# Autodesk Inventor assembly: Turret ASM
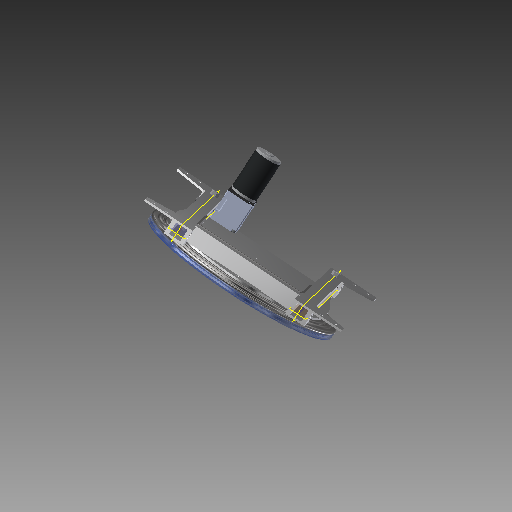
[picture p0: Inventor's stored thumbnail of the model, 512x512]
Saved by Autodesk Inventor 2017 (Build 210142000, 142)
## iProperties
Created: 2016-09-26
Part Number: Turret ASM
Document SubType Name: Assembly
Designer: Hanson
Author: Hanson
## Documents named in this file (19)
- C:\Users\Thariq\Documents\GitHub\bps-bunnybots2016-cad\bps-bunnybots2016-cad\Bunnybot-To_be_renamed\15102898-16-A-0000\15102898-16-A-0600\Turret ASM.iam
- C:\Users\Thariq\Documents\GitHub\bps-bunnybots2016-cad\bps-bunnybots2016-cad\Bunnybot-To_be_renamed\15102898-16-A-0000\15102898-16-A-0600\User Library-LazySusan 12inch.ipt
- C:\Users\Thariq\Documents\GitHub\bps-bunnybots2016-cad\bps-bunnybots2016-cad\Bunnybot-To_be_renamed\15102898-16-A-0000\15102898-16-A-0600\Large crossbeam.ipt
- C:\Users\Thariq\Documents\GitHub\bps-bunnybots2016-cad\bps-bunnybots2016-cad\Bunnybot-To_be_renamed\15102898-16-A-0000\15102898-16-A-0600\90480A195_LOW-STRENGTH STEEL HEX NUT.ipt
- C:\Users\Thariq\Documents\GitHub\bps-bunnybots2016-cad\bps-bunnybots2016-cad\Bunnybot-To_be_renamed\15102898-16-A-0000\15102898-16-A-0600\92196A277_18-8 STAINLESS STEEL SOCKET HEAD CAP SCREW.ipt
- C:\Users\Thariq\Documents\GitHub\bps-bunnybots2016-cad\bps-bunnybots2016-cad\Bunnybot-To_be_renamed\15102898-16-A-0000\15102898-16-A-0600\BAG motor top plate.ipt
- C:\Users\Thariq\Documents\GitHub\bps-bunnybots2016-cad\bps-bunnybots2016-cad\Bunnybot-To_be_renamed\15102898-16-A-0000\15102898-16-A-0600\92196A545_18-8 STAINLESS STEEL SOCKET HEAD CAP SCREW.ipt
- C:\Users\Thariq\Documents\GitHub\bps-bunnybots2016-cad\bps-bunnybots2016-cad\Bunnybot-To_be_renamed\15102898-16-A-0000\15102898-16-A-0600\plate mount nut.ipt
- C:\Users\Thariq\Documents\GitHub\bps-bunnybots2016-cad\bps-bunnybots2016-cad\Bunnybot-To_be_renamed\15102898-16-A-0000\15102898-16-A-0600\lazy susan bushing.ipt
- C:\Users\Thariq\Documents\GitHub\bps-bunnybots2016-cad\bps-bunnybots2016-cad\Bunnybot-To_be_renamed\15102898-16-A-0000\15102898-16-A-0600\BAG motor\VersaPlanetary-1-Stage-with-BAG-Motor.iam
- C:\Users\Thariq\Documents\GitHub\bps-bunnybots2016-cad\bps-bunnybots2016-cad\Bunnybot-To_be_renamed\15102898-16-A-0000\15102898-16-A-0600\217-2642-STEP-20140807.ipt
- C:\Users\Thariq\Documents\GitHub\bps-bunnybots2016-cad\bps-bunnybots2016-cad\Bunnybot-To_be_renamed\15102898-16-A-0000\15102898-16-A-0600\support ring.ipt
- C:\Users\Thariq\Documents\GitHub\bps-bunnybots2016-cad\bps-bunnybots2016-cad\Bunnybot-To_be_renamed\15102898-16-A-0000\15102898-16-A-0600\roundplate.ipt
- C:\Users\Thariq\Documents\GitHub\bps-bunnybots2016-cad\bps-bunnybots2016-cad\Bunnybot-To_be_renamed\15102898-16-A-0000\15102898-16-A-0600\Turret ASM\Design Accelerator\Chain Drive3.iam
- C:\Users\Thariq\Documents\GitHub\bps-bunnybots2016-cad\bps-bunnybots2016-cad\Bunnybot-To_be_renamed\15102898-16-A-0000\15102898-16-A-0200\Imported Components\1556A170_BRACKET.ipt
- C:\Users\Thariq\Documents\GitHub\bps-bunnybots2016-cad\bps-bunnybots2016-cad\Bunnybot-To_be_renamed\15102898-16-A-0000\15102898-16-A-0600\horizontal bar.ipt
- C:\Users\Thariq\Documents\GitHub\bps-bunnybots2016-cad\bps-bunnybots2016-cad\Bunnybot-To_be_renamed\15102898-16-A-0000\15102898-16-A-0600\2x1 angle bracket.ipt
- C:\Users\Thariq\Documents\GitHub\bps-bunnybots2016-cad\bps-bunnybots2016-cad\Bunnybot-To_be_renamed\15102898-16-A-0000\15102898-16-A-0600\15102898-16-P-0207.ipt
- C:\Users\Thariq\Documents\GitHub\bps-bunnybots2016-cad\bps-bunnybots2016-cad\Bunnybot-To_be_renamed\15102898-16-A-0000\15102898-16-A-0600\15102898-16-P-0208.ipt
## Components (27 placed, 18 different names)
1. User Library-LazySusan 12inch:1 — Mate:5, Mate:7, Mate:10, Mate:25, Mate:26, Mate:27, Mate:28, Mate:29
2. Large crossbeam:1 — Insert:16, Flush:1, Flush:2, Mate:17, Flush:3, Mate:34, Mate:35, Flush:10, Mate:41, Flush:14, Flush:17, Mate:43, Flush:18, Mate:44, Flush:19, Flush:20
3. Large crossbeam:2 — Insert:13, Insert:14, Insert:15, Flush:1, Mate:14, Flush:2, Mate:19, Flush:6, Flush:8, Flush:9, Mate:37, Flush:11, Mate:39, Flush:12, Mate:42, Flush:15, Flush:16, Flush:21, Mate:45, Flush:22
4. 92196A277_18-8 STAINLESS STEEL SOCKET HEAD CAP SCREW:1 — Insert:13
5. 92196A277_18-8 STAINLESS STEEL SOCKET HEAD CAP SCREW:2 — Insert:14
6. BAG motor top plate:1 — Insert:11, Insert:12, Mate:14, Flush:3, Mate:18, Flush:4, Flush:6, Mate:25, Mate:26, Mate:27, Mate:30
7. 92196A545_18-8 STAINLESS STEEL SOCKET HEAD CAP SCREW:1 — Insert:11
8. 92196A545_18-8 STAINLESS STEEL SOCKET HEAD CAP SCREW:2 — Insert:12, Mate:17
9. plate mount nut:1 — Insert:15
10. plate mount nut:2 — Insert:16
11. lazy susan bushing:1 — Mate:5, Mate:24
12. 90480A195_LOW-STRENGTH STEEL HEX NUT:2 — Mate:7, Mate:24
13. 90480A195_LOW-STRENGTH STEEL HEX NUT:4 — Mate:10
14. VersaPlanetary-1-Stage-with-BAG-Motor:1 [sub-assembly] — Mate:18, Mate:19, Flush:4, Mate:20, Mate:21
15. 217-2642-STEP-20140807:1 — Mate:20, Mate:21, Flush:7
16. support ring:1 — Mate:28, Mate:29, Mate:30, Mate:31, Mate:32, Mate:33
17. roundplate:1 — Mate:31, Mate:32, Mate:33, Flush:7
18. Chain Drive:1 [sub-assembly]
19. 1556A170_BRACKET:1 — Mate:37, Mate:38, Flush:11
20. 1556A170_BRACKET:2 — Mate:35, Mate:36, Flush:10
21. horizontal bar:1 — Mate:34, Flush:8, Flush:9, Mate:36, Mate:38, Mate:40
22. 2x1 angle bracket:1 — Mate:39, Mate:40, Flush:12, Flush:13
23. 2x1 angle bracket:2 — Flush:13, Mate:41, Flush:14
24. 15102898-16-P-0207:1 — Flush:17, Mate:43, Flush:18
25. 15102898-16-P-0208:1 — Mate:42, Flush:15, Flush:16
26. 15102898-16-P-0207:2 — Flush:21, Mate:45, Flush:22
27. 15102898-16-P-0208:2 — Mate:44, Flush:19, Flush:20
## Relationships (58: Mate 31, Flush 21, Insert 6)
- Insert:11: BAG motor top plate:1 ↔ 92196A545_18-8 STAINLESS STEEL SOCKET HEAD CAP SCREW:1
- Insert:12: BAG motor top plate:1 ↔ 92196A545_18-8 STAINLESS STEEL SOCKET HEAD CAP SCREW:2
- Insert:13: Large crossbeam:2 ↔ 92196A277_18-8 STAINLESS STEEL SOCKET HEAD CAP SCREW:1
- Insert:14: Large crossbeam:2 ↔ 92196A277_18-8 STAINLESS STEEL SOCKET HEAD CAP SCREW:2
- Insert:15: Large crossbeam:2 ↔ plate mount nut:1
- Insert:16: Large crossbeam:1 ↔ plate mount nut:2
- Flush:1: Large crossbeam:1 ↔ Large crossbeam:2
- Mate:5: User Library-LazySusan 12inch:1 ↔ lazy susan bushing:1
- Mate:7: User Library-LazySusan 12inch:1 ↔ 90480A195_LOW-STRENGTH STEEL HEX NUT:2
- Mate:10: User Library-LazySusan 12inch:1 ↔ 90480A195_LOW-STRENGTH STEEL HEX NUT:4
- Mate:14: Large crossbeam:2 ↔ BAG motor top plate:1
- Flush:2: Large crossbeam:1 ↔ Large crossbeam:2
- Mate:17: Large crossbeam:1 ↔ 92196A545_18-8 STAINLESS STEEL SOCKET HEAD CAP SCREW:2
- Flush:3: Large crossbeam:1 ↔ BAG motor top plate:1
- Mate:18: BAG motor top plate:1 ↔ VersaPlanetary-1-Stage-with-BAG-Motor:1
- Mate:19: Large crossbeam:2 ↔ VersaPlanetary-1-Stage-with-BAG-Motor:1
- Flush:4: BAG motor top plate:1 ↔ VersaPlanetary-1-Stage-with-BAG-Motor:1
- Mate:20: VersaPlanetary-1-Stage-with-BAG-Motor:1 ↔ 217-2642-STEP-20140807:1
- Mate:21: VersaPlanetary-1-Stage-with-BAG-Motor:1 ↔ 217-2642-STEP-20140807:1
- Mate:24: lazy susan bushing:1 ↔ 90480A195_LOW-STRENGTH STEEL HEX NUT:2
- Flush:6: Large crossbeam:2 ↔ BAG motor top plate:1
- Mate:25: User Library-LazySusan 12inch:1 ↔ BAG motor top plate:1
- Mate:26: User Library-LazySusan 12inch:1 ↔ BAG motor top plate:1
- Mate:27: User Library-LazySusan 12inch:1 ↔ BAG motor top plate:1
- Mate:28: User Library-LazySusan 12inch:1 ↔ support ring:1
- Mate:29: User Library-LazySusan 12inch:1 ↔ support ring:1
- Mate:30: BAG motor top plate:1 ↔ support ring:1
- Mate:31: support ring:1 ↔ roundplate:1
- Mate:32: support ring:1 ↔ roundplate:1
- Mate:33: support ring:1 ↔ roundplate:1
- Flush:7: 217-2642-STEP-20140807:1 ↔ roundplate:1
- Mate:34: Large crossbeam:1 ↔ horizontal bar:1
- Flush:8: Large crossbeam:2 ↔ horizontal bar:1
- Flush:9 (50.8 mm): Large crossbeam:2 ↔ horizontal bar:1
- Mate:35: Large crossbeam:1 ↔ 1556A170_BRACKET:2
- Mate:36: 1556A170_BRACKET:2 ↔ horizontal bar:1
- Flush:10: Large crossbeam:1 ↔ 1556A170_BRACKET:2
- Mate:37: Large crossbeam:2 ↔ 1556A170_BRACKET:1
- Mate:38: 1556A170_BRACKET:1 ↔ horizontal bar:1
- Flush:11: Large crossbeam:2 ↔ 1556A170_BRACKET:1
- Mate:39: Large crossbeam:2 ↔ 2x1 angle bracket:1
- Mate:40: horizontal bar:1 ↔ 2x1 angle bracket:1
- Flush:12: Large crossbeam:2 ↔ 2x1 angle bracket:1
- Flush:13: 2x1 angle bracket:1 ↔ 2x1 angle bracket:2
- Mate:41: Large crossbeam:1 ↔ 2x1 angle bracket:2
- Flush:14: Large crossbeam:1 ↔ 2x1 angle bracket:2
- Mate:42: Large crossbeam:2 ↔ 15102898-16-P-0208:1
- Flush:15: Large crossbeam:2 ↔ 15102898-16-P-0208:1
- Flush:16: Large crossbeam:2 ↔ 15102898-16-P-0208:1
- Flush:17: Large crossbeam:1 ↔ 15102898-16-P-0207:1
- Mate:43: Large crossbeam:1 ↔ 15102898-16-P-0207:1
- Flush:18: Large crossbeam:1 ↔ 15102898-16-P-0207:1
- Mate:44: Large crossbeam:1 ↔ 15102898-16-P-0208:2
- Flush:19: Large crossbeam:1 ↔ 15102898-16-P-0208:2
- Flush:20: Large crossbeam:1 ↔ 15102898-16-P-0208:2
- Flush:21: Large crossbeam:2 ↔ 15102898-16-P-0207:2
- Mate:45: Large crossbeam:2 ↔ 15102898-16-P-0207:2
- Flush:22: Large crossbeam:2 ↔ 15102898-16-P-0207:2
